# Autodesk Inventor assembly: Caisson
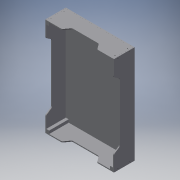
[picture p0: Inventor's stored thumbnail of the model, 180x180]
Saved by Autodesk Inventor 2016 SP1 (Build 200210100, 210)
## iProperties
Created: 2017-04-26
Part Number: Caisson
Material: Générique
Document SubType Name: Assembly
Designer: dimercur
Author: dimercur
## Documents named in this file (7)
- D:\Users\dimercur\Documents\git\dev-gei\dev-gei2\Circuit-a-Bille\Caisson.iam
- D:\Users\dimercur\Documents\git\dev-gei\dev-gei2\Circuit-a-Bille\Coté long plateau - 2.ipt
- D:\Users\dimercur\Documents\git\dev-gei\dev-gei2\Circuit-a-Bille\Coté long plateau -1.ipt
- D:\Users\dimercur\Documents\git\dev-gei\dev-gei2\Circuit-a-Bille\Coté court plateau.ipt
- D:\Users\dimercur\Documents\git\dev-gei\dev-gei2\Circuit-a-Bille\Tasseau-1.ipt
- D:\Users\dimercur\Documents\git\dev-gei\dev-gei2\Circuit-a-Bille\Plateau.ipt
- D:\Users\dimercur\Documents\Inventor\Content Center Files\R2016\fr-FR\ISO 7045  H\ISO 7045 - M2,5 x 6 - 4.8 - H - ISO.ipt
## Components (35 placed, 5 different names)
1. Coté long plateau:1 — Placage:6, Placage:8, Placage:9, Placage:12, Placage:13, Logement:1, Logement:2, Logement:3, Logement:4
2. Coté long plateau:2 — Placage:5, Placage:7, Placage:10, Placage:11, Placage:14, Placage:19, Placage:20, Logement:9, Logement:10, Logement:11, Logement:12
3. Coté court plateau:1 — Placage:15, Placage:17, Placage:20, Placage:21, Placage:22, Logement:5, Logement:6, Logement:7, Logement:8
4. Coté court plateau:2 — Placage:16, Placage:18, Placage:19, Placage:23, Placage:24, Logement:13, Logement:14, Logement:15, Logement:16
5. Tasseau-1:1 — Placage:4, Placage:13, Placage:23
6. Tasseau-1:2 — Placage:3, Placage:14, Placage:24
7. Tasseau-1:3 — Placage:2, Placage:11, Placage:21
8. Tasseau-1:4 — Placage:1, Placage:12, Placage:22
9. Plateau:1 — Placage:1, Placage:2, Placage:3, Placage:4, Placage:5, Placage:6, Placage:7, Placage:8, Placage:9, Placage:10, Placage:15, Placage:16, Placage:17, Placage:18, Logement:17, Logement:18, Logement:19, Logement:20, Logement:21, Logement:22, Logement:23, Logement:24, Logement:25, Logement:26
10. ISO 7045 H M2,5 x 6 - 4.8 - H:1 — Logement:1
11. ISO 7045 H M2,5 x 6 - 4.8 - H:2 — Logement:2
12. ISO 7045 H M2,5 x 6 - 4.8 - H:3 — Logement:3
13. ISO 7045 H M2,5 x 6 - 4.8 - H:4 — Logement:4
14. ISO 7045 H M2,5 x 6 - 4.8 - H:5 — Logement:5
15. ISO 7045 H M2,5 x 6 - 4.8 - H:6 — Logement:6
16. ISO 7045 H M2,5 x 6 - 4.8 - H:7 — Logement:7
17. ISO 7045 H M2,5 x 6 - 4.8 - H:8 — Logement:8
18. ISO 7045 H M2,5 x 6 - 4.8 - H:9 — Logement:9
19. ISO 7045 H M2,5 x 6 - 4.8 - H:10 — Logement:10
20. ISO 7045 H M2,5 x 6 - 4.8 - H:11 — Logement:11
21. ISO 7045 H M2,5 x 6 - 4.8 - H:12 — Logement:12
22. ISO 7045 H M2,5 x 6 - 4.8 - H:13 — Logement:13
23. ISO 7045 H M2,5 x 6 - 4.8 - H:14 — Logement:14
24. ISO 7045 H M2,5 x 6 - 4.8 - H:15 — Logement:15
25. ISO 7045 H M2,5 x 6 - 4.8 - H:16 — Logement:16
26. ISO 7045 H M2,5 x 6 - 4.8 - H:17 — Logement:17
27. ISO 7045 H M2,5 x 6 - 4.8 - H:18 — Logement:18
28. ISO 7045 H M2,5 x 6 - 4.8 - H:19 — Logement:19
29. ISO 7045 H M2,5 x 6 - 4.8 - H:20 — Logement:20
30. ISO 7045 H M2,5 x 6 - 4.8 - H:21 — Logement:21
31. ISO 7045 H M2,5 x 6 - 4.8 - H:22 — Logement:22
32. ISO 7045 H M2,5 x 6 - 4.8 - H:23 — Logement:23
33. ISO 7045 H M2,5 x 6 - 4.8 - H:24 — Logement:24
34. ISO 7045 H M2,5 x 6 - 4.8 - H:25 — Logement:25
35. ISO 7045 H M2,5 x 6 - 4.8 - H:26 — Logement:26
## Relationships (50: Insert 26, Mate 24)
- Placage:1 [Mate]: Tasseau-1:4 ↔ Plateau:1
- Placage:2 [Mate]: Tasseau-1:3 ↔ Plateau:1
- Placage:3 [Mate]: Tasseau-1:2 ↔ Plateau:1
- Placage:4 [Mate]: Tasseau-1:1 ↔ Plateau:1
- Placage:5 [Mate]: Coté long plateau:2 ↔ Plateau:1
- Placage:6 [Mate]: Coté long plateau:1 ↔ Plateau:1
- Placage:7 [Mate]: Coté long plateau:2 ↔ Plateau:1
- Placage:8 [Mate]: Coté long plateau:1 ↔ Plateau:1
- Placage:9 [Mate]: Coté long plateau:1 ↔ Plateau:1
- Placage:10 [Mate]: Coté long plateau:2 ↔ Plateau:1
- Placage:11 [Mate]: Coté long plateau:2 ↔ Tasseau-1:3
- Placage:12 [Mate]: Coté long plateau:1 ↔ Tasseau-1:4
- Placage:13 [Mate]: Coté long plateau:1 ↔ Tasseau-1:1
- Placage:14 [Mate]: Coté long plateau:2 ↔ Tasseau-1:2
- Placage:15 [Mate]: Coté court plateau:1 ↔ Plateau:1
- Placage:16 [Mate]: Coté court plateau:2 ↔ Plateau:1
- Placage:17 [Mate]: Coté court plateau:1 ↔ Plateau:1
- Placage:18 [Mate]: Coté court plateau:2 ↔ Plateau:1
- Placage:19 [Mate]: Coté long plateau:2 ↔ Coté court plateau:2
- Placage:20 [Mate]: Coté long plateau:2 ↔ Coté court plateau:1
- Placage:21 [Mate]: Coté court plateau:1 ↔ Tasseau-1:3
- Placage:22 [Mate]: Coté court plateau:1 ↔ Tasseau-1:4
- Placage:23 [Mate]: Coté court plateau:2 ↔ Tasseau-1:1
- Placage:24 [Mate]: Coté court plateau:2 ↔ Tasseau-1:2
- Logement:1 [Insert]: Coté long plateau:1 ↔ ISO 7045 H M2,5 x 6 - 4.8 - H:1
- Logement:2 [Insert]: Coté long plateau:1 ↔ ISO 7045 H M2,5 x 6 - 4.8 - H:2
- Logement:3 [Insert]: Coté long plateau:1 ↔ ISO 7045 H M2,5 x 6 - 4.8 - H:3
- Logement:4 [Insert]: Coté long plateau:1 ↔ ISO 7045 H M2,5 x 6 - 4.8 - H:4
- Logement:5 [Insert]: Coté court plateau:1 ↔ ISO 7045 H M2,5 x 6 - 4.8 - H:5
- Logement:6 [Insert]: Coté court plateau:1 ↔ ISO 7045 H M2,5 x 6 - 4.8 - H:6
- Logement:7 [Insert]: Coté court plateau:1 ↔ ISO 7045 H M2,5 x 6 - 4.8 - H:7
- Logement:8 [Insert]: Coté court plateau:1 ↔ ISO 7045 H M2,5 x 6 - 4.8 - H:8
- Logement:9 [Insert]: Coté long plateau:2 ↔ ISO 7045 H M2,5 x 6 - 4.8 - H:9
- Logement:10 [Insert]: Coté long plateau:2 ↔ ISO 7045 H M2,5 x 6 - 4.8 - H:10
- Logement:11 [Insert]: Coté long plateau:2 ↔ ISO 7045 H M2,5 x 6 - 4.8 - H:11
- Logement:12 [Insert]: Coté long plateau:2 ↔ ISO 7045 H M2,5 x 6 - 4.8 - H:12
- Logement:13 [Insert]: Coté court plateau:2 ↔ ISO 7045 H M2,5 x 6 - 4.8 - H:13
- Logement:14 [Insert]: Coté court plateau:2 ↔ ISO 7045 H M2,5 x 6 - 4.8 - H:14
- Logement:15 [Insert]: Coté court plateau:2 ↔ ISO 7045 H M2,5 x 6 - 4.8 - H:15
- Logement:16 [Insert]: Coté court plateau:2 ↔ ISO 7045 H M2,5 x 6 - 4.8 - H:16
- Logement:17 [Insert]: Plateau:1 ↔ ISO 7045 H M2,5 x 6 - 4.8 - H:17
- Logement:18 [Insert]: Plateau:1 ↔ ISO 7045 H M2,5 x 6 - 4.8 - H:18
- Logement:19 [Insert]: Plateau:1 ↔ ISO 7045 H M2,5 x 6 - 4.8 - H:19
- Logement:20 [Insert]: Plateau:1 ↔ ISO 7045 H M2,5 x 6 - 4.8 - H:20
- Logement:21 [Insert]: Plateau:1 ↔ ISO 7045 H M2,5 x 6 - 4.8 - H:21
- Logement:22 [Insert]: Plateau:1 ↔ ISO 7045 H M2,5 x 6 - 4.8 - H:22
- Logement:23 [Insert]: Plateau:1 ↔ ISO 7045 H M2,5 x 6 - 4.8 - H:23
- Logement:24 [Insert]: Plateau:1 ↔ ISO 7045 H M2,5 x 6 - 4.8 - H:24
- Logement:25 [Insert]: Plateau:1 ↔ ISO 7045 H M2,5 x 6 - 4.8 - H:25
- Logement:26 [Insert]: Plateau:1 ↔ ISO 7045 H M2,5 x 6 - 4.8 - H:26
